# Autodesk Inventor assembly: wheel_shock
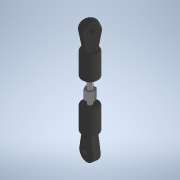
[picture p0: Inventor's stored thumbnail of the model, 180x180]
Saved by Autodesk Inventor 2020 (Build 240168000, 168)
## iProperties
Created: 2020-03-09
Part Number: wheel_shock
Document SubType Name: Assembly
Designer: 0x6f736f646f
Author: 0x6f736f646f
## Documents named in this file (3)
- C:\Users\0x6f736f646f\Documents\Inventor\Eureka_Autonomous_CAR\wheel_shock.iam
- C:\Users\0x6f736f646f\Documents\Inventor\Eureka_Autonomous_CAR\wheel_shock_pin.ipt
- C:\Users\0x6f736f646f\Documents\Inventor\Eureka_Autonomous_CAR\wheel_shock_end.ipt
## Components (3 placed, 2 different names)
1. wheel_shock_pin:1 — Mate:1, Mate:2
2. wheel_shock_end:1 — Mate:1
3. wheel_shock_end:2 — Mate:2
## Relationships (2: Mate 2)
- Mate:1: wheel_shock_pin:1 ↔ wheel_shock_end:1
- Mate:2: wheel_shock_pin:1 ↔ wheel_shock_end:2
